# Autodesk Inventor assembly: Battery
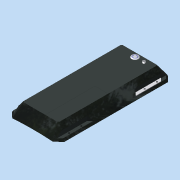
[picture p0: Inventor's stored thumbnail of the model, 180x180]
Saved by Autodesk Inventor 2015 (Build 190159000, 159)
## iProperties
Created: 2015-12-28
Part Number: Battery
Document SubType Name: Assembly
Designer: Raphael
Author: Raphael
## Documents named in this file (7)
- \\psf\Home\Documents\electric-skateboard\CAD\Battery.iam
- \\psf\Home\Documents\electric-skateboard\CAD\BatteryEnclosure.ipt
- \\psf\Home\Documents\electric-skateboard\CAD\BatteryPack.iam
- \\psf\Home\Documents\electric-skateboard\CAD\BatteryHeatsink.ipt
- \\psf\Home\Documents\electric-skateboard\CAD\BMS.ipt
- \\psf\Home\Documents\electric-skateboard\CAD\Vandal Resistant Switch.iam
- \\psf\Home\Documents\electric-skateboard\CAD\pj-065b.iam
## Components (6 placed, 6 different names)
1. BatteryEnclosure:1 — Mate:1, Mate:2, Mate:3, Mate:4, Mate:5, Mate:6, Mate:7, Mate:8, Mate:9, Mate:10, Mate:11, Tangent:3, Tangent:4
2. BatteryPack:1 [sub-assembly] — Mate:4, Tangent:3, Tangent:4
3. BatteryHeatsink:1 — Mate:1, Mate:2, Mate:3
4. BMS:1 — Mate:5, Mate:6, Mate:7
5. Vandal Resistant Switch:1 [sub-assembly] — Mate:8, Mate:9
6. pj-065b:1 [sub-assembly] — Mate:10, Mate:11
## Relationships (13: Mate 11, Tangent 2)
- Mate:1: BatteryEnclosure:1 ↔ BatteryHeatsink:1
- Mate:2: BatteryEnclosure:1 ↔ BatteryHeatsink:1
- Mate:3: BatteryEnclosure:1 ↔ BatteryHeatsink:1
- Mate:4: BatteryEnclosure:1 ↔ BatteryPack:1
- Mate:5: BatteryEnclosure:1 ↔ BMS:1
- Mate:6: BatteryEnclosure:1 ↔ BMS:1
- Mate:7: BatteryEnclosure:1 ↔ BMS:1
- Mate:8: BatteryEnclosure:1 ↔ Vandal Resistant Switch:1
- Mate:9: BatteryEnclosure:1 ↔ Vandal Resistant Switch:1
- Mate:10: BatteryEnclosure:1 ↔ pj-065b:1
- Mate:11: BatteryEnclosure:1 ↔ pj-065b:1
- Tangent:3: BatteryEnclosure:1 ↔ BatteryPack:1
- Tangent:4: BatteryEnclosure:1 ↔ BatteryPack:1
